# Autodesk Inventor assembly: Sliders
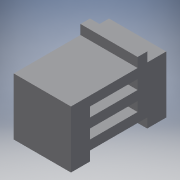
[picture p0: Inventor's stored thumbnail of the model, 180x180]
Saved by Autodesk Inventor 2016 (Build 200138000, 138)
## iProperties
Created: 2012-03-04
Part Number: Sliders
Document SubType Name: Assembly
Designer: John
Author: John
## Documents named in this file (2)
- C:\File Storage\Autodesk\Inventor 2016 Projects\Ex_Files_Inventor_2016_EssT\Exercise Files\15_Using constraints to position parts\15_07\Sliders.iam
- C:\File Storage\Autodesk\Inventor 2016 Projects\Ex_Files_Inventor_2016_EssT\Exercise Files\15_Using constraints to position parts\15_07\Slider.ipt
## Components (3 placed, 1 different names)
1. Slider:1 — Mate:1, Flush:1, Flush:3 DRIVE THIS
2. Slider:2 — Mate:1, Flush:1, Mate:2, Flush:2
3. Slider:3 — Mate:2, Flush:2, Flush:3 DRIVE THIS
## Relationships (5: Flush 3, Mate 2)
- Mate:1: Slider:1 ↔ Slider:2
- Flush:1: Slider:1 ↔ Slider:2
- Mate:2: Slider:2 ↔ Slider:3
- Flush:2: Slider:2 ↔ Slider:3
- Flush:3 DRIVE THIS: Slider:1 ↔ Slider:3
